# Autodesk Inventor assembly: Upper_Deck
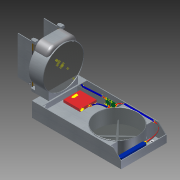
[picture p0: Inventor's stored thumbnail of the model, 180x180]
Saved by Autodesk Inventor 2011 SP1 (Build 150282100, 282)
## iProperties
Created: 2011-05-30
Part Number: Upper_Deck
Document SubType Name: Assembly
Designer: Andrew G. Meyer
Mass: 2188.08 g
Surface Area: 13831.5 cm^2
Volume: 2188.08 cm^3
Density: 1 g/cm^3
Author: Andrew G. Meyer
## Documents named in this file (26)
- C:\Users\Andrew G. Meyer\Documents\Inventor\Hovercraft\CAD\Upper_Deck.iam
- C:\Users\Andrew G. Meyer\Documents\Inventor\Hovercraft\CAD\Side_Panel.ipt
- C:\Users\Andrew G. Meyer\Documents\Inventor\Hovercraft\CAD\Base_Panel.ipt
- C:\Users\Andrew G. Meyer\Documents\Inventor\Hovercraft\CAD\Lift_Duct.iam
- C:\Users\Andrew G. Meyer\Documents\Inventor\Hovercraft\CAD\Duct_Support.ipt
- C:\Users\Andrew G. Meyer\Documents\Inventor\Hovercraft\CAD\Thrust_Duct.iam
- C:\Users\Andrew G. Meyer\Documents\Inventor\Hovercraft\CAD\Aft_Panel.ipt
- C:\Users\Andrew G. Meyer\Documents\Inventor\Hovercraft\CAD\Aft_Top.ipt
- C:\Users\Andrew G. Meyer\Documents\Inventor\Hovercraft\CAD\Front.ipt
- C:\Users\Andrew G. Meyer\Documents\Inventor\Hovercraft\CAD\Fore_Top.ipt
- C:\Users\Andrew G. Meyer\Documents\Inventor\Hovercraft\CAD\Upper_Rudder_Duct_Support.ipt
- C:\Users\Andrew G. Meyer\Documents\Inventor\Hovercraft\CAD\Rudder_Bracket.ipt
- C:\Users\Andrew G. Meyer\Documents\Inventor\Hovercraft\CAD\Rudder_Hinge_Pin.ipt
- C:\Users\Andrew G. Meyer\Documents\Inventor\Hovercraft\CAD\Port_Rudder.iam
- C:\Users\Andrew G. Meyer\Documents\Inventor\Hovercraft\CAD\Starboard_Rudder.iam
- C:\Users\Andrew G. Meyer\Documents\Inventor\Hovercraft\CAD\Rudder_Link.ipt
- C:\Users\Andrew G. Meyer\Documents\Inventor\Hovercraft\CAD\Aft_Support.ipt
- C:\Users\Andrew G. Meyer\Documents\Inventor\Hovercraft\CAD\Deck_Nut.ipt
- C:\Users\Andrew G. Meyer\Documents\Inventor\Hovercraft\CAD\Upper_Deck\AIP\Cable and Harness\Thrust_Harness.iam
- C:\Users\Andrew G. Meyer\Documents\Inventor\Hovercraft\CAD\xM.ipt
- C:\Users\Andrew G. Meyer\Documents\Inventor\Hovercraft\CAD\Battery.ipt
- C:\Users\Andrew G. Meyer\Documents\Inventor\Hovercraft\CAD\Duct_Support_Cut.ipt
- C:\Users\Andrew G. Meyer\Documents\Inventor\Hovercraft\CAD\PDU.ipt
- C:\Users\Andrew G. Meyer\Documents\Inventor\Hovercraft\CAD\Upper_Deck\AIP\Cable and Harness\Battery_Line.iam
- C:\Users\Andrew G. Meyer\Documents\Inventor\Hovercraft\CAD\Upper_Deck\AIP\Cable and Harness\Thrust_Power.iam
- C:\Users\Andrew G. Meyer\Documents\Inventor\Hovercraft\CAD\Upper_Deck\AIP\Cable and Harness\xM_Power.iam
## Components (37 placed, 25 different names)
1. Side_Panel:1 — Mate:2, Flush:1, Flush:2, Mate:4, Mate:13, Mate:15, Mate:21, Mate:34, Mate:41
2. Side_Panel:2 — Mate:1, Flush:3, Mate:11, Mate:14, Mate:16, Flush:9, Mate:20, Mate:35, Mate:38, Mate:45, Mate:47, Flush:23
3. Base_Panel:1 — Mate:1, Mate:2, Flush:1, Flush:2, Insert:1, Mate:6, Flush:3, Flush:6, Mate:12, Flush:7, Mate:19, Flush:10, Flush:11, Insert:11, Insert:12, Insert:13, Insert:14, Insert:15, Insert:16, Mate:36, Mate:43, Mate:46
4. Lift_Duct:1 [sub-assembly] — Insert:1, Mate:39, Mate:44
5. Duct_Support:1 — Mate:4, Mate:6, Mate:39
6. Duct_Support:3 — Mate:11, Flush:6, Insert:2, Mate:18, Flush:13, Flush:14, Flush:18, Flush:19, Flush:22
7. Thrust_Duct:1 [sub-assembly] — Insert:2, Mate:23
8. Aft_Panel:1 — Mate:12, Mate:13, Mate:14, Flush:7, Mate:17, Flush:8, Mate:32, Mate:33, Mate:37
9. Aft_Top:1 — Mate:15, Mate:16, Mate:17, Flush:8, Mate:18, Mate:22, Flush:12, Mate:30, Mate:31
10. Front:1 — Mate:19, Flush:9, Flush:10, Flush:11, Mate:42
11. Fore_Top:1 — Mate:20, Mate:21, Mate:22, Flush:12
12. Upper_Rudder_Duct_Support:1 — Flush:13, Flush:14, Mate:23, Mate:26, Flush:17, Mate:28, Flush:21
13. Rudder_Bracket:1 — Insert:4, Flush:15, Mate:28, Flush:21, Mate:29
14. Rudder_Bracket:2 — Insert:5, Flush:15, Flush:22
15. Rudder_Bracket:3 — Insert:7, Flush:16, Mate:26, Flush:17, Insert:8, Mate:27, Flush:20
16. Rudder_Bracket:4 — Flush:16, Flush:18, Flush:19, Flush:20
17. Rudder_Hinge_Pin:1 — Insert:4, Mate:24, Insert:5
18. Rudder_Hinge_Pin:2 — Mate:25, Insert:7, Insert:8
19. Port_Rudder:1 [sub-assembly] — Mate:24, Mate:29, Insert:9
20. Starboard_Rudder:1 [sub-assembly] — Mate:25, Mate:27, Insert:10
21. Rudder_Link:1 — Insert:9, Insert:10
22. Aft_Support:1 — Mate:30, Mate:33, Mate:34
23. Aft_Support:2 — Mate:31, Mate:32, Mate:35
24. Deck_Nut:1 — Insert:13
25. Deck_Nut:2 — Insert:12
26. Deck_Nut:3 — Insert:14
27. Deck_Nut:4 — Insert:11
28. Deck_Nut:5 — Insert:16
29. Deck_Nut:6 — Insert:15
30. Thrust_Harness [sub-assembly]
31. xM:1 — Mate:36, Mate:37, Mate:38
32. Battery:1 — Mate:41, Mate:42, Mate:43
33. Duct_Support_Cut:1 — Mate:44, Mate:45, Mate:46, Mate:48
34. PDU:1 — Mate:47, Mate:48, Flush:23
35. Battery_Line [sub-assembly]
36. Thrust_Power [sub-assembly]
37. xM_Power [sub-assembly]
## Relationships (76: Mate 41, Flush 21, Insert 14)
- Mate:1: Side_Panel:2 ↔ Base_Panel:1
- Mate:2: Side_Panel:1 ↔ Base_Panel:1
- Flush:1: Side_Panel:1 ↔ Base_Panel:1
- Flush:2: Side_Panel:1 ↔ Base_Panel:1
- Insert:1: Base_Panel:1 ↔ Lift_Duct:1
- Mate:4: Side_Panel:1 ↔ Duct_Support:1
- Mate:6: Base_Panel:1 ↔ Duct_Support:1
- Flush:3: Side_Panel:2 ↔ Base_Panel:1
- Mate:11 (38.1 mm): Side_Panel:2 ↔ Duct_Support:3
- Flush:6 (-25.4 mm): Base_Panel:1 ↔ Duct_Support:3
- Insert:2: Duct_Support:3 ↔ Thrust_Duct:1
- Mate:12: Base_Panel:1 ↔ Aft_Panel:1
- Mate:13: Side_Panel:1 ↔ Aft_Panel:1
- Mate:14: Side_Panel:2 ↔ Aft_Panel:1
- Flush:7: Base_Panel:1 ↔ Aft_Panel:1
- Mate:15: Side_Panel:1 ↔ Aft_Top:1
- Mate:16: Side_Panel:2 ↔ Aft_Top:1
- Mate:17: Aft_Panel:1 ↔ Aft_Top:1
- Flush:8: Aft_Panel:1 ↔ Aft_Top:1
- Mate:18: Duct_Support:3 ↔ Aft_Top:1
- Mate:19: Base_Panel:1 ↔ Front:1
- Flush:9: Side_Panel:2 ↔ Front:1
- Flush:10: Base_Panel:1 ↔ Front:1
- Flush:11: Base_Panel:1 ↔ Front:1
- Mate:20: Side_Panel:2 ↔ Fore_Top:1
- Mate:21: Side_Panel:1 ↔ Fore_Top:1
- Mate:22: Aft_Top:1 ↔ Fore_Top:1
- Flush:12: Aft_Top:1 ↔ Fore_Top:1
- Flush:13: Duct_Support:3 ↔ Upper_Rudder_Duct_Support:1
- Flush:14: Duct_Support:3 ↔ Upper_Rudder_Duct_Support:1
- Mate:23: Thrust_Duct:1 ↔ Upper_Rudder_Duct_Support:1
- Insert:4: Rudder_Bracket:1 ↔ Rudder_Hinge_Pin:1
- Mate:24: Rudder_Hinge_Pin:1 ↔ Port_Rudder:1
- Insert:5: Rudder_Bracket:2 ↔ Rudder_Hinge_Pin:1
- Flush:15: Rudder_Bracket:1 ↔ Rudder_Bracket:2
- Mate:25: Rudder_Hinge_Pin:2 ↔ Starboard_Rudder:1
- Insert:7: Rudder_Bracket:3 ↔ Rudder_Hinge_Pin:2
- Flush:16: Rudder_Bracket:3 ↔ Rudder_Bracket:4
- Mate:26: Upper_Rudder_Duct_Support:1 ↔ Rudder_Bracket:3
- Flush:17: Upper_Rudder_Duct_Support:1 ↔ Rudder_Bracket:3
- Insert:8: Rudder_Bracket:3 ↔ Rudder_Hinge_Pin:2
- Mate:27 (1.5875 mm): Rudder_Bracket:3 ↔ Starboard_Rudder:1
- Flush:18: Duct_Support:3 ↔ Rudder_Bracket:4
- Flush:19: Duct_Support:3 ↔ Rudder_Bracket:4
- Flush:20: Rudder_Bracket:3 ↔ Rudder_Bracket:4
- Mate:28: Upper_Rudder_Duct_Support:1 ↔ Rudder_Bracket:1
- Flush:21: Upper_Rudder_Duct_Support:1 ↔ Rudder_Bracket:1
- Flush:22: Duct_Support:3 ↔ Rudder_Bracket:2
- Mate:29 (1.5875 mm): Rudder_Bracket:1 ↔ Port_Rudder:1
- Insert:9: Port_Rudder:1 ↔ Rudder_Link:1
- Insert:10: Starboard_Rudder:1 ↔ Rudder_Link:1
- Mate:30: Aft_Top:1 ↔ Aft_Support:1
- Mate:31: Aft_Top:1 ↔ Aft_Support:2
- Mate:32: Aft_Panel:1 ↔ Aft_Support:2
- Mate:33: Aft_Panel:1 ↔ Aft_Support:1
- Mate:34: Side_Panel:1 ↔ Aft_Support:1
- Mate:35: Side_Panel:2 ↔ Aft_Support:2
- Insert:11: Base_Panel:1 ↔ Deck_Nut:4
- Insert:12: Base_Panel:1 ↔ Deck_Nut:2
- Insert:13: Base_Panel:1 ↔ Deck_Nut:1
- Insert:14: Base_Panel:1 ↔ Deck_Nut:3
- Insert:15: Base_Panel:1 ↔ Deck_Nut:6
- Insert:16: Base_Panel:1 ↔ Deck_Nut:5
- Mate:36: Base_Panel:1 ↔ xM:1
- Mate:37 (12.7 mm): Aft_Panel:1 ↔ xM:1
- Mate:38: Side_Panel:2 ↔ xM:1
- Mate:39: Lift_Duct:1 ↔ Duct_Support:1
- Mate:41: Side_Panel:1 ↔ Battery:1
- Mate:42: Front:1 ↔ Battery:1
- Mate:43: Base_Panel:1 ↔ Battery:1
- Mate:44: Lift_Duct:1 ↔ Duct_Support_Cut:1
- Mate:45: Side_Panel:2 ↔ Duct_Support_Cut:1
- Mate:46: Base_Panel:1 ↔ Duct_Support_Cut:1
- Mate:47: Side_Panel:2 ↔ PDU:1
- Mate:48 (38.1 mm): Duct_Support_Cut:1 ↔ PDU:1
- Flush:23 (25.4 mm): Side_Panel:2 ↔ PDU:1
